# Autodesk Inventor assembly: holder_2021
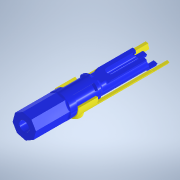
[picture p0: Inventor's stored thumbnail of the model, 180x180]
Saved by Autodesk Inventor 2021 (Build 250183000, 183)
## iProperties
Created: 2021-02-05
Part Number: holder_2021
Document SubType Name: Assembly
Designer: dsdan
Author: dsdan
## Documents named in this file (3)
- E:\OneDrive - Imperial College London\DragonVision_DanielKo\Instrumentation\Ephys_rig_2021\Holder\holder_2021.iam
- E:\OneDrive - Imperial College London\DragonVision_DanielKo\Instrumentation\Ephys_rig_2021\Holder\body_adjustable_v4_sympetrum.ipt
- E:\OneDrive - Imperial College London\DragonVision_DanielKo\Instrumentation\Ephys_rig_2021\Holder\head_adjustable_v3.ipt
## Components (2 placed, 2 different names)
1. body_adjustable_v4_sympetrum:1 — Mate:4, Mate:2, Flush:1, Mate:3
2. head_adjustable_v3:1 — Mate:4, Mate:2
## Relationships (4: Mate 3, Flush 1)
- Mate:4: body_adjustable_v4_sympetrum:1 ↔ head_adjustable_v3:1
- Mate:2: body_adjustable_v4_sympetrum:1 ↔ head_adjustable_v3:1
- Flush:1: body_adjustable_v4_sympetrum:1
- Mate:3: body_adjustable_v4_sympetrum:1
